# Autodesk Inventor assembly: BarcoFinal
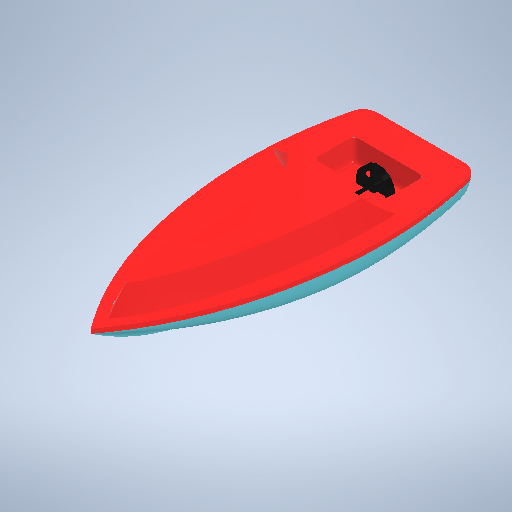
[picture p0: Inventor's stored thumbnail of the model, 512x512]
Saved by Autodesk Inventor 2025.2 (Build 292293000, 293)
## iProperties
Created: 2025-02-27
Part Number: BarcoFinal
Document SubType Name: Assembly
Designer: yovan
Author: yovan
## Documents named in this file (5)
- C:\Users\usuario\Documents\GitHub\ausol-apm.github.io\project\Design and simulation\Inventor\Modelado juguetes\Barco\BarcoFinal.iam
- C:\Users\usuario\Documents\GitHub\ausol-apm.github.io\project\Design and simulation\Inventor\Modelado juguetes\Barco\Inferior.ipt
- C:\Users\usuario\Documents\GitHub\ausol-apm.github.io\project\Design and simulation\Inventor\Modelado juguetes\Barco\Piezabarcosuperior.ipt
- C:\Users\usuario\Documents\GitHub\ausol-apm.github.io\project\Design and simulation\Inventor\Modelado juguetes\Barco\PiezaTimon.ipt
- C:\Users\usuario\Documents\GitHub\ausol-apm.github.io\project\Design and simulation\Inventor\Modelado juguetes\Barco\Timon.ipt
## Components (4 placed, 4 different names)
1. Inferior:1 — Coincidencia:4, Coincidencia:5, Coincidencia:6
2. Piezabarcosuperior:1 — Coincidencia:1, Coincidencia:2, Coincidencia:3, Coincidencia:4, Coincidencia:5, Coincidencia:6
3. PiezaTimon:1 — Insertar:1
4. Timon:1 — Insertar:1, Coincidencia:1, Coincidencia:2, Coincidencia:3
## Relationships (7: Mate 6, Insert 1)
- Insertar:1: PiezaTimon:1 ↔ Timon:1
- Coincidencia:1 [Mate]: Piezabarcosuperior:1 ↔ Timon:1
- Coincidencia:2 [Mate]: Piezabarcosuperior:1 ↔ Timon:1
- Coincidencia:3 [Mate]: Piezabarcosuperior:1 ↔ Timon:1
- Coincidencia:4 [Mate]: Inferior:1 ↔ Piezabarcosuperior:1
- Coincidencia:5 [Mate]: Inferior:1 ↔ Piezabarcosuperior:1
- Coincidencia:6 [Mate]: Inferior:1 ↔ Piezabarcosuperior:1
